# Autodesk Inventor assembly: 上半身
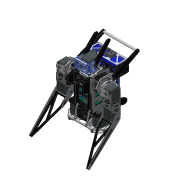
[picture p0: Inventor's stored thumbnail of the model, 180x180]
Saved by Autodesk Inventor 2016 (Build 200138000, 138)
## iProperties
Created: 2016-05-03
Part Number: 上半身
Document SubType Name: Assembly
Designer: hiroaki
Mass: 2009.19 g
Surface Area: 5971.27 cm^2
Volume: 1067.53 cm^3
Density: 1.88209 g/cm^3
Author: hiroaki
## Documents named in this file (5)
- C:\Users\haya\Desktop\OpenPlatform\上半身.iam
- C:\Users\haya\Desktop\OpenPlatform\上半身\胴体\胴体_1.iam
- C:\Users\haya\Desktop\OpenPlatform\上半身\腕\上腕_1.iam
- C:\Users\haya\Desktop\OpenPlatform\上半身\腕\前腕_1.iam
- C:\Users\haya\Desktop\OpenPlatform\上半身\腕\肩_1.iam
## Components (7 placed, 4 different names)
1. 胴体_1:1 [sub-assembly] — 挿入:5, 角度:1, 挿入:8, 角度:5, 角度:8, 角度:9
2. 上腕_1:1 [sub-assembly] — 挿入:1, 挿入:3, 挿入:4, 角度:1, 角度:2, 角度:3, 角度:5, 角度:6, 角度:7, 角度:8, 角度:9
3. 前腕_1:1 [sub-assembly] — 挿入:1, 角度:3, 角度:4, 角度:6
4. 肩_1:1 [sub-assembly] — 挿入:3, 挿入:4, 挿入:5
5. 肩_1:2 [sub-assembly] — 挿入:7, 挿入:8
6. 上腕_1:2 [sub-assembly] — 挿入:7, 角度:2, 角度:7, 挿入:9
7. 前腕_1:2 [sub-assembly] — 角度:4, 挿入:9
## Relationships (16: Angle 9, Insert 7)
- 挿入:1 [Insert]: 上腕_1:1 ↔ 前腕_1:1
- 挿入:3 [Insert]: 上腕_1:1 ↔ 肩_1:1
- 挿入:4 [Insert]: 上腕_1:1 ↔ 肩_1:1
- 挿入:5 [Insert]: 胴体_1:1 ↔ 肩_1:1
- 角度:1 [Angle] (0 deg): 胴体_1:1 ↔ 上腕_1:1
- 挿入:7 [Insert]: 肩_1:2 ↔ 上腕_1:2
- 挿入:8 [Insert]: 胴体_1:1 ↔ 肩_1:2
- 角度:2 [Angle] (0 deg): 上腕_1:1 ↔ 上腕_1:2
- 角度:3 [Angle] (45 deg): 上腕_1:1 ↔ 前腕_1:1
- 角度:4 [Angle] (0 deg): 前腕_1:1 ↔ 前腕_1:2
- 角度:5 [Angle] (0 deg): 胴体_1:1 ↔ 上腕_1:1
- 角度:6 [Angle] (-90 deg): 上腕_1:1 ↔ 前腕_1:1
- 角度:7 [Angle] (0 deg): 上腕_1:1 ↔ 上腕_1:2
- 挿入:9 [Insert]: 上腕_1:2 ↔ 前腕_1:2
- 角度:8 [Angle] (0 deg): 胴体_1:1 ↔ 上腕_1:1
- 角度:9 [Angle] (0 deg): 胴体_1:1 ↔ 上腕_1:1
